# Autodesk Inventor assembly: 204.006.01_ZB_Extrudereinheit
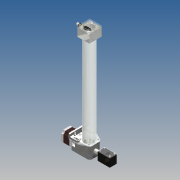
[picture p0: Inventor's stored thumbnail of the model, 180x180]
Saved by Autodesk Inventor 2021 (Build 250183000, 183)
## iProperties
Created: 2021-12-04
Part Number: 204.006.01_ZB_Extrudereinheit
Document SubType Name: Assembly
Designer: Sebastian Seewald
Author: Sebastian Seewald
## Documents named in this file (4)
- E:\Dokumente\MCI-Mechatronik\Master\Semester_3\Projekt_2_Neu\104_Extrudereinheit\204.006.01_ZB_Extrudereinheit.iam
- E:\Dokumente\MCI-Mechatronik\Master\Semester_3\Projekt_2_Neu\104_Extrudereinheit\204.003.01_ZB_Extruder.iam
- E:\Dokumente\MCI-Mechatronik\Master\Semester_3\Projekt_2_Neu\104_Extrudereinheit\204.002.01_ZB_Fuehlstandsmessung.iam
- E:\Dokumente\MCI-Mechatronik\Master\Semester_3\Projekt_2_Neu\104_Extrudereinheit\104.010.01_Zwischenstueck_oben.ipt
## Components (3 placed, 3 different names)
1. 204.003.01_ZB_Extruder:1 [sub-assembly] — Passend:1, Passend:2, Winkel:1
2. 204.002.01_ZB_Fuehlstandsmessung:1 [sub-assembly] — Passend:1, Passend:2, Winkel:1, Passend:3, Passend:4, Passend:5
3. 104.010.01_Zwischenstueck_oben:1 — Passend:3, Passend:4, Passend:5
## Relationships (6: Mate 5, Angle 1)
- Passend:1 [Mate]: 204.003.01_ZB_Extruder:1 ↔ 204.002.01_ZB_Fuehlstandsmessung:1
- Passend:2 [Mate]: 204.003.01_ZB_Extruder:1 ↔ 204.002.01_ZB_Fuehlstandsmessung:1
- Winkel:1 [Angle] (0 deg): 204.003.01_ZB_Extruder:1 ↔ 204.002.01_ZB_Fuehlstandsmessung:1
- Passend:3 [Mate]: 204.002.01_ZB_Fuehlstandsmessung:1 ↔ 104.010.01_Zwischenstueck_oben:1
- Passend:4 [Mate]: 204.002.01_ZB_Fuehlstandsmessung:1 ↔ 104.010.01_Zwischenstueck_oben:1
- Passend:5 [Mate]: 204.002.01_ZB_Fuehlstandsmessung:1 ↔ 104.010.01_Zwischenstueck_oben:1
